# Autodesk Inventor assembly: 000-3p-robot-v1
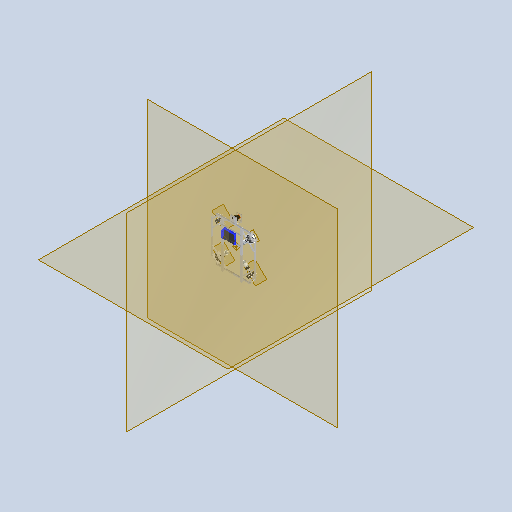
[picture p0: Inventor's stored thumbnail of the model, 512x512]
Saved by Autodesk Inventor 2025.2 (Build 292293000, 293)
## iProperties
Created: 2024-10-24
Part Number: 000-3p-robot-v1
Document SubType Name: Assembly
Designer: haruy
Mass: 34983.9 g
Surface Area: 44613.1 cm^2
Volume: 13427.3 cm^3
Density: 2.60542 g/cm^3
Author: haruy
## Documents named in this file (3)
- C:\Users\haruy\Documents\ロボコン\NHK2025\cad\nagahisa\gazebo\3p-robot-v1.iam
- C:\Users\haruy\Documents\ロボコン\NHK2025\cad\nagahisa\base_weel\takagi_weel\Workspaces\作業スペース\takagi\omuni_wheel_ver3.0\omuni_wheel_ver3.0.iam
- C:\Users\haruy\Documents\ロボコン\NHK2025\cad\nagahisa\dribl\R2-Rzvector\000-RZvector-v1.iam
## Components (2 placed, 2 different names)
1. omuni_wheel_ver3.0:1 [sub-assembly] — 挿入:1, 挿入:2, 角度:3, フラッシュ:1, フラッシュ:2, メイト:1
2. 000-RZvector-v1:1 [sub-assembly] — 挿入:1, 挿入:2
## Relationships (6: Insert 2, Flush 2, Angle 1, Mate 1)
- 挿入:1 [Insert]: omuni_wheel_ver3.0:1 ↔ 000-RZvector-v1:1
- 挿入:2 [Insert]: omuni_wheel_ver3.0:1 ↔ 000-RZvector-v1:1
- 角度:3 [Angle] (0 deg): omuni_wheel_ver3.0:1
- フラッシュ:1 [Flush] (52.428 mm): omuni_wheel_ver3.0:1
- フラッシュ:2 [Flush] (-315 mm): omuni_wheel_ver3.0:1
- メイト:1 [Mate] (-315 mm): omuni_wheel_ver3.0:1
